# Autodesk Inventor assembly: Tote Collector Arm_MIR1
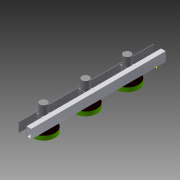
[picture p0: Inventor's stored thumbnail of the model, 180x180]
Saved by Autodesk Inventor 2015 (Build 190159000, 159)
## iProperties
Created: 2015-01-11
Part Number: Tote Collector Arm_MIR1
Document SubType Name: Assembly
Designer: chapale16
Author: chapale16
## Documents named in this file (5)
- \\lhssvr02\Homedirs\Robotics Club\CAD Model 2015\Game Components\The Tote Collector-Arms\Tote Collector Arm_MIR1.iam
- \\lhssvr02\Homedirs\Robotics Club\CAD Model 2015\Game Components\The Tote Collector-Arms\P60 Gear Box_MIR1.ipt
- \\lhssvr02\Homedirs\Robotics Club\CAD Model 2015\Game Components\The Tote Collector-Arms\Arm_MIR1.ipt
- \\lhssvr02\Homedirs\Robotics Club\CAD Model 2015\Game Components\The Tote Collector-Arms\collector arm wheel_MIR1.ipt
- \\lhssvr02\Homedirs\Robotics Club\CAD Model 2015\Game Components\The Tote Collector-Arms\Sheet Metal side_MIR.ipt
## Components (8 placed, 4 different names)
1. P60 Gear Box_MIR1:1 — Flush:5, Flush:1, Mate:4
2. P60 Gear Box_MIR1:2 — Flush:6, Flush:2, Mate:5
3. P60 Gear Box_MIR1:3 — Flush:4, Flush:3, Mate:6, Mate:7
4. Arm_MIR1:1 — Flush:6, Flush:5, Flush:4, Flush:8, Flush:7
5. collector arm wheel_MIR1:1 — Flush:3, Mate:6
6. collector arm wheel_MIR1:2 — Flush:2, Mate:5
7. collector arm wheel_MIR1:3 — Flush:1, Mate:4
8. Sheet Metal side_MIR:1 — Flush:8, Flush:7, Mate:7
## Relationships (12: Flush 8, Mate 4)
- Flush:6: P60 Gear Box_MIR1:2 ↔ Arm_MIR1:1
- Flush:5: P60 Gear Box_MIR1:1 ↔ Arm_MIR1:1
- Flush:4: P60 Gear Box_MIR1:3 ↔ Arm_MIR1:1
- Flush:3: P60 Gear Box_MIR1:3 ↔ collector arm wheel_MIR1:1
- Mate:6: P60 Gear Box_MIR1:3 ↔ collector arm wheel_MIR1:1
- Flush:2: P60 Gear Box_MIR1:2 ↔ collector arm wheel_MIR1:2
- Mate:5: P60 Gear Box_MIR1:2 ↔ collector arm wheel_MIR1:2
- Flush:1: P60 Gear Box_MIR1:1 ↔ collector arm wheel_MIR1:3
- Mate:4: P60 Gear Box_MIR1:1 ↔ collector arm wheel_MIR1:3
- Flush:8: Arm_MIR1:1 ↔ Sheet Metal side_MIR:1
- Flush:7: Arm_MIR1:1 ↔ Sheet Metal side_MIR:1
- Mate:7: P60 Gear Box_MIR1:3 ↔ Sheet Metal side_MIR:1
